# Autodesk Inventor assembly: Overall_Shooting_Mechanism2
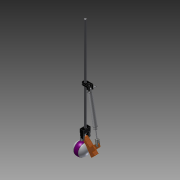
[picture p0: Inventor's stored thumbnail of the model, 180x180]
Saved by Autodesk Inventor 2015 (Build 190159000, 159)
## iProperties
Created: 2017-02-21
Part Number: Overall_Shooting_Mechanism2
Document SubType Name: Assembly
Designer: Guy
Author: Guy
## Documents named in this file (11)
- C:\Users\Guy\Documents\Fourth Year\Capstone\git\Capstone-Project\doc\CAD\SM2\Overall_Shooting_Mechanism2.iam
- C:\Users\Guy\Documents\Fourth Year\Capstone\git\Capstone-Project\doc\CAD\SM2\Swinging_connection.ipt
- C:\Users\Guy\Documents\Fourth Year\Capstone\git\Capstone-Project\doc\CAD\SM2\hinge_for_swing.ipt
- C:\Users\Guy\Documents\Fourth Year\Capstone\git\Capstone-Project\doc\CAD\SM2\Piston_Holder.ipt
- C:\Users\Guy\Documents\Fourth Year\Capstone\git\Capstone-Project\doc\CAD\SM2\Small_piston.ipt
- C:\Users\Guy\Documents\Fourth Year\Capstone\git\Capstone-Project\doc\CAD\SM2\piston_rod_connector.ipt
- C:\Users\Guy\Documents\Fourth Year\Capstone\git\Capstone-Project\doc\CAD\SM2\piston_internal_rod.ipt
- C:\Users\Guy\Documents\Fourth Year\Capstone\git\Capstone-Project\doc\CAD\LowLevel_Rev2\Pool_Ball_Stripe.ipt
- C:\Users\Guy\Documents\Fourth Year\Capstone\git\Capstone-Project\doc\CAD\SM2\1-2in_eebase_connector.ipt
- C:\Users\Guy\Documents\Fourth Year\Capstone\git\Capstone-Project\doc\CAD\Nuts and Bolts\3-16in_1 1-4in_Bolt.ipt
- C:\Users\Guy\Documents\Fourth Year\Capstone\git\Capstone-Project\doc\CAD\Nuts and Bolts\3-16in_1-16in_nut(num2).ipt
## Components (12 placed, 10 different names)
1. 1-2in_eebase_connector:1 — Mate:35, Mate:36, Angle:1, Flush:6
2. hinge_for_swing:2 — Mate:29, Mate:32, Mate:34, Mate:36, Angle:1, Flush:6, Mate:37, Mate:38, Mate:39
3. Pool_Ball_Stripe:1
4. Piston_Holder:1 — Mate:26, Mate:29, Mate:30, Mate:35, Mate:41, Mate:42, Mate:43, Mate:44
5. piston_internal_rod:1 — Mate:21, Mate:22, Flush:5
6. piston_rod_connector:1 — Mate:21, Flush:5, Mate:31, Mate:33
7. Small_piston:1 — Mate:22, Mate:26, Mate:30, Mate:31
8. Swinging_connection:1 — Mate:32, Mate:33, Mate:34
9. 3-16in_1 1-4in_Bolt:1 — Mate:37, Mate:38, Mate:40
10. 3-16in_1-16in_nut(num2):1 — Mate:39, Mate:40
11. 3-16in_1 1-4in_Bolt:2 — Mate:43, Mate:44
12. 3-16in_1-16in_nut(num2):2 — Mate:41, Mate:42
## Relationships (22: Mate 19, Flush 2, Angle 1)
- Mate:21: piston_internal_rod:1 ↔ piston_rod_connector:1
- Mate:22: piston_internal_rod:1 ↔ Small_piston:1
- Flush:5: piston_internal_rod:1 ↔ piston_rod_connector:1
- Mate:26: Piston_Holder:1 ↔ Small_piston:1
- Mate:29 (170 mm): hinge_for_swing:2 ↔ Piston_Holder:1
- Mate:30 (1 mm): Piston_Holder:1 ↔ Small_piston:1
- Mate:31 (37.8 mm): piston_rod_connector:1 ↔ Small_piston:1
- Mate:32: hinge_for_swing:2 ↔ Swinging_connection:1
- Mate:33: piston_rod_connector:1 ↔ Swinging_connection:1
- Mate:34 (0.5 mm): hinge_for_swing:2 ↔ Swinging_connection:1
- Mate:35: 1-2in_eebase_connector:1 ↔ Piston_Holder:1
- Mate:36: 1-2in_eebase_connector:1 ↔ hinge_for_swing:2
- Angle:1 (0 deg): 1-2in_eebase_connector:1 ↔ hinge_for_swing:2
- Flush:6 (8 mm): 1-2in_eebase_connector:1 ↔ hinge_for_swing:2
- Mate:37: hinge_for_swing:2 ↔ 3-16in_1 1-4in_Bolt:1
- Mate:38: hinge_for_swing:2 ↔ 3-16in_1 1-4in_Bolt:1
- Mate:39: hinge_for_swing:2 ↔ 3-16in_1-16in_nut(num2):1
- Mate:40: 3-16in_1 1-4in_Bolt:1 ↔ 3-16in_1-16in_nut(num2):1
- Mate:41: Piston_Holder:1 ↔ 3-16in_1-16in_nut(num2):2
- Mate:42: Piston_Holder:1 ↔ 3-16in_1-16in_nut(num2):2
- Mate:43: Piston_Holder:1 ↔ 3-16in_1 1-4in_Bolt:2
- Mate:44: Piston_Holder:1 ↔ 3-16in_1 1-4in_Bolt:2
